# Autodesk Inventor assembly: WELDMENT,ARM
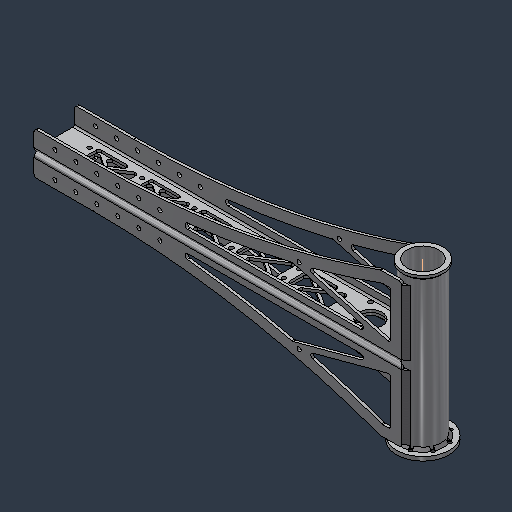
[picture p0: Inventor's stored thumbnail of the model, 512x512]
Saved by Autodesk Inventor 2024.3 (Build 283343000, 343)
## iProperties
Category: _
Manager: _
Created: 2025-03-12
Part Number: WELDMENT,ARM
Checked By: 00
Engr Approved By: _
User Status: Work In Process
Description: Weldment (ANSI)
Document SubType Name: Weldment
Mfg Approved By: John.Thibert
Designer: John.Thibert
Weld Material: Welded Steel Mild
Mass: 911.543 g
Surface Area: 2357.06 cm^2
Volume: 330.713 cm^3
CN_MASS: 0.85
CN_SERVICEABLE: _
CL_runCount: 0
FIRST_DESCRIPTION: _
SECOND_DESCRIPTION: _
THIRD_DESCRIPTION: _
ModelCat: Uncategorized
ILogicPurgeVersion: 2.2.20.20
OnSaveVersion: 3.5.0.0
OnSaveAssembly: COREAutomationManager
Subject: _
Author: John.Thibert
Keywords: -
Revision Number: -
## Documents named in this file (4)
- D:\Inventor Projects\Poseidon V2\WELDMENT,ARM.iam
- D:\Inventor Projects\Poseidon V2\TUBE,1.5IN,ARM.ipt
- D:\Inventor Projects\Poseidon V2\PLATE,TOP,ARM,DG.ipt
- D:\Inventor Projects\Poseidon V2\HUB,GEAR,ARM.ipt
## Components (4 placed, 3 different names)
1. PLATE,TOP,ARM,DG:2 — Mate:5, Mate:7, Flush:7
2. PLATE,TOP,ARM,DG:1 — Mate:6, Flush:6, Mate:8
3. TUBE,1.5IN,ARM:1 — Flush:5, Mate:4, Mate:5, Mate:6, Mate:7, Flush:8
4. HUB,GEAR,ARM:1
## Relationships (11: Mate 7, Flush 4)
- Flush:5: TUBE,1.5IN,ARM:1
- Mate:4: TUBE,1.5IN,ARM:1
- Mate:5: PLATE,TOP,ARM,DG:2 ↔ TUBE,1.5IN,ARM:1
- Mate:6: PLATE,TOP,ARM,DG:1 ↔ TUBE,1.5IN,ARM:1
- Flush:6: PLATE,TOP,ARM,DG:1
- Mate:7: PLATE,TOP,ARM,DG:2 ↔ TUBE,1.5IN,ARM:1
- Mate:8: PLATE,TOP,ARM,DG:1
- Flush:7: PLATE,TOP,ARM,DG:2
- Flush:8: TUBE,1.5IN,ARM:1
- [Mate]: TUBE,1.5IN,ARM:1 ↔ HUB,GEAR,ARM:1
- [Mate]: PLATE,TOP,ARM,DG:2 ↔ HUB,GEAR,ARM:1
